# Autodesk Inventor assembly: Corpo_Suspensao_Cabos
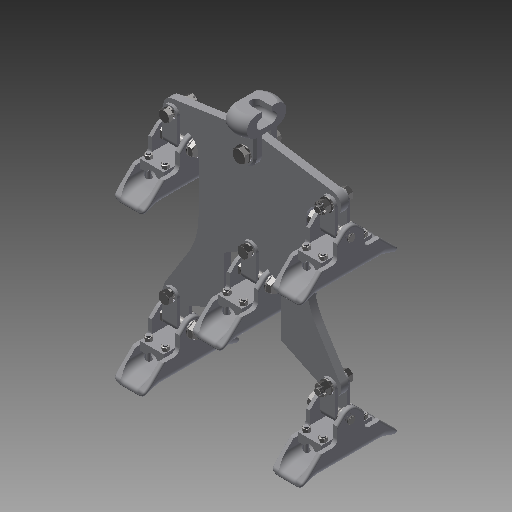
[picture p0: Inventor's stored thumbnail of the model, 512x512]
Saved by Autodesk Inventor 2018 (Build 220112000, 112)
## iProperties
Created: 2021-04-28
Part Number: Corpo_Suspensao_Cabos
Document SubType Name: Assembly
Designer: l01767
Author: l01767
## Documents named in this file (4)
- F:\Projetos\TAESA\Modelo 3D - Tensionadores e Suspensão\Suporte de Suspenção\Corpo_Suspensao_Cabos.iam
- F:\Projetos\TAESA\Modelo 3D - Tensionadores e Suspensão\Suporte de Suspenção\Corpo_Suporte_Cabos.ipt
- F:\Projetos\TAESA\Modelo 3D - Tensionadores e Suspensão\Suporte de Suspenção\Clevis-Socket.iam
- F:\Projetos\TAESA\Modelo 3D - Tensionadores e Suspensão\Suporte de Suspenção\Suspenssion_Clamp.iam
## Components (7 placed, 3 different names)
1. Corpo_Suporte_Cabos:1 — Mate:1, Flush:1, Mate:2, Mate:3, Mate:4, Mate:5, Mate:7, Mate:9
2. Clevis-Socket:1 [sub-assembly] — Mate:3, Mate:4, Angle:1
3. Suspenssion_Clamp:5 [sub-assembly] — Mate:7, Mate:8
4. Suspenssion_Clamp:1 [sub-assembly] — Mate:5, Mate:6, Angle:2, Angle:3
5. Suspenssion_Clamp:2 [sub-assembly] — Mate:9, Flush:2, Angle:3
6. Suspenssion_Clamp:6 [sub-assembly]
7. Suspenssion_Clamp:7 [sub-assembly]
## Component patterns: (2 elements, first: Suspenssion_Clamp:1 + Suspenssion_Clamp:2)
## Relationships (14: Mate 9, Angle 3, Flush 2)
- Mate:1: Corpo_Suporte_Cabos:1
- Flush:1: Corpo_Suporte_Cabos:1
- Mate:2: Corpo_Suporte_Cabos:1
- Mate:3: Corpo_Suporte_Cabos:1 ↔ Clevis-Socket:1
- Mate:4: Corpo_Suporte_Cabos:1 ↔ Clevis-Socket:1
- Angle:1 (0 deg): Clevis-Socket:1
- Mate:5: Corpo_Suporte_Cabos:1 ↔ Suspenssion_Clamp:1
- Mate:6: Suspenssion_Clamp:1
- Angle:2 (0 deg): Suspenssion_Clamp:1
- Mate:7: Corpo_Suporte_Cabos:1 ↔ Suspenssion_Clamp:5
- Mate:8: Suspenssion_Clamp:5
- Mate:9: Corpo_Suporte_Cabos:1 ↔ Suspenssion_Clamp:2
- Flush:2: Suspenssion_Clamp:2
- Angle:3 (180 deg): Suspenssion_Clamp:1 ↔ Suspenssion_Clamp:2
